# Autodesk Inventor assembly: Body_Assembly
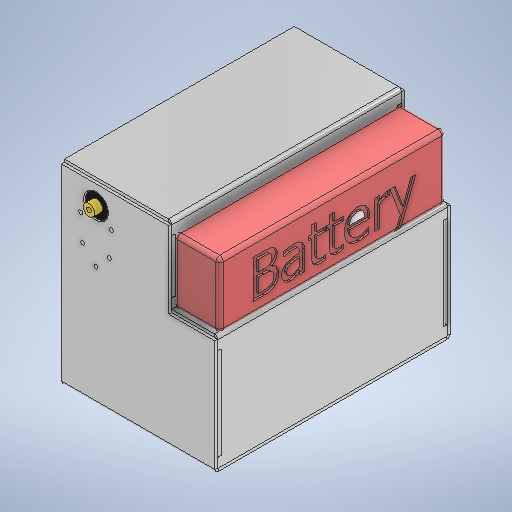
[picture p0: Inventor's stored thumbnail of the model, 512x512]
Saved by Autodesk Inventor 2025.2 (Build 292293000, 293)
## iProperties
Created: 2025-05-07
Part Number: Body_Assembly
Document SubType Name: Assembly
Designer: chris
Author: chris
## Documents named in this file (12)
- C:\Users\chris\문서\Inventor\RHp_Humanoid_ver1\Assembly\1_Body.iam
- C:\Users\chris\문서\Inventor\RHp_Humanoid_ver1\Part\Frame\Body\body_main_frame.ipt
- C:\Users\chris\문서\Inventor\RHp_Humanoid_ver1\Part\Frame\Body\body_front_frame.ipt
- C:\Users\chris\문서\Inventor\RHp_Humanoid_ver1\Part\Frame\Body\body_middle_frame.ipt
- C:\Users\chris\문서\Inventor\RHp_Humanoid_ver1\Part\Frame\Body\body_back_frame.ipt
- C:\Users\chris\문서\Inventor\RHp_Humanoid_ver1\Part\Frame\Body\body_motor_R_frame.ipt
- C:\Users\chris\문서\Inventor\RHp_Humanoid_ver1\Part\HTD-45H, Horn\HTD-45H\HTD-45H.iam
- C:\Users\chris\문서\Inventor\RHp_Humanoid_ver1\Part\HTD-45H, Horn\HTD-45H\HTD-45H.ipt
- C:\Users\chris\문서\Inventor\RHp_Humanoid_ver1\Part\Frame\Body\body_top_frame.ipt
- C:\Users\chris\문서\Inventor\RHp_Humanoid_ver1\Part\Frame\Body\Battery_Pack.ipt
- C:\Users\chris\문서\Inventor\P3766-P3768SKU4-P3767ENVELOPE\jetson_orin_super.iam
- C:\Users\chris\문서\Inventor\RHp_Humanoid_ver1\Part\Frame\Body\Servo_Driver.ipt
## Components (12 placed, 10 different names)
1. body_main_frame:1 — Mate:1, Mate:2, Mate:3, Mate:4, Flush:1, Mate:5, Mate:6, Flush:3, Mate:7, Mate:8, Flush:4, Mate:10, Mate:14, Mate:17, Mate:18, Flush:9, Flush:10, Mate:22, Flush:11, Mate:23, Flush:12
2. body_front_frame:1 — Mate:1, Mate:2, Mate:3, Flush:2, Mate:9, Flush:5, Mate:13
3. body_middle_frame:1 — Flush:2, Mate:6, Flush:3, Mate:11, Flush:6, Flush:7, Mate:15, Flush:8, Mate:21, Mate:24
4. body_back_frame:1 — Mate:7, Mate:8, Flush:4, Mate:20
5. body_motor_R_frame:1 — Mate:9, Flush:5, Mate:12
6. HTD-45H:1 [sub-assembly] — Mate:10, Flush:6, Mate:11, Mate:12
7. body_motor_R_frame:2 — Mate:13, Flush:7, Mate:16
8. HTD-45H:2 — Mate:14, Mate:15, Flush:8, Mate:16
9. body_top_frame:1 — Mate:17, Mate:18, Flush:9, Mate:19
10. Battery_Pack:1 — Mate:19, Mate:20, Flush:10
11. jetson_orin_super:1 [sub-assembly] — Mate:21, Mate:22, Flush:11
12. Servo_Driver:1 — Mate:23, Mate:24, Flush:12
## Relationships (36: Mate 24, Flush 12)
- Mate:1: body_main_frame:1 ↔ body_front_frame:1
- Mate:2: body_main_frame:1 ↔ body_front_frame:1
- Mate:3 (1.5 mm): body_main_frame:1 ↔ body_front_frame:1
- Mate:4: body_main_frame:1
- Flush:1: body_main_frame:1
- Mate:5: body_main_frame:1
- Flush:2 (30 mm): body_front_frame:1 ↔ body_middle_frame:1
- Mate:6: body_main_frame:1 ↔ body_middle_frame:1
- Flush:3: body_main_frame:1 ↔ body_middle_frame:1
- Mate:7: body_main_frame:1 ↔ body_back_frame:1
- Mate:8: body_main_frame:1 ↔ body_back_frame:1
- Flush:4: body_main_frame:1 ↔ body_back_frame:1
- Mate:9: body_front_frame:1 ↔ body_motor_R_frame:1
- Flush:5: body_front_frame:1 ↔ body_motor_R_frame:1
- Mate:10: body_main_frame:1 ↔ HTD-45H:1
- Flush:6: body_middle_frame:1 ↔ HTD-45H:1
- Mate:11 (2 mm): body_middle_frame:1 ↔ HTD-45H:1
- Mate:12: body_motor_R_frame:1 ↔ HTD-45H:1
- Mate:13: body_front_frame:1 ↔ body_motor_R_frame:2
- Flush:7: body_middle_frame:1 ↔ body_motor_R_frame:2
- Mate:14: body_main_frame:1 ↔ HTD-45H:2
- Mate:15 (2 mm): body_middle_frame:1 ↔ HTD-45H:2
- Flush:8: body_middle_frame:1 ↔ HTD-45H:2
- Mate:16: body_motor_R_frame:2 ↔ HTD-45H:2
- Mate:17: body_main_frame:1 ↔ body_top_frame:1
- Mate:18: body_main_frame:1 ↔ body_top_frame:1
- Flush:9: body_main_frame:1 ↔ body_top_frame:1
- Mate:19: body_top_frame:1 ↔ Battery_Pack:1
- Mate:20: body_back_frame:1 ↔ Battery_Pack:1
- Flush:10 (-2.5 mm): body_main_frame:1 ↔ Battery_Pack:1
- Mate:21: body_middle_frame:1 ↔ jetson_orin_super:1
- Mate:22: body_main_frame:1 ↔ jetson_orin_super:1
- Flush:11 (10 mm): body_main_frame:1 ↔ jetson_orin_super:1
- Mate:23: body_main_frame:1 ↔ Servo_Driver:1
- Mate:24: body_middle_frame:1 ↔ Servo_Driver:1
- Flush:12 (32.5 mm): body_main_frame:1 ↔ Servo_Driver:1
